# Autodesk Inventor assembly: LIDAR-Mapping-Assembly
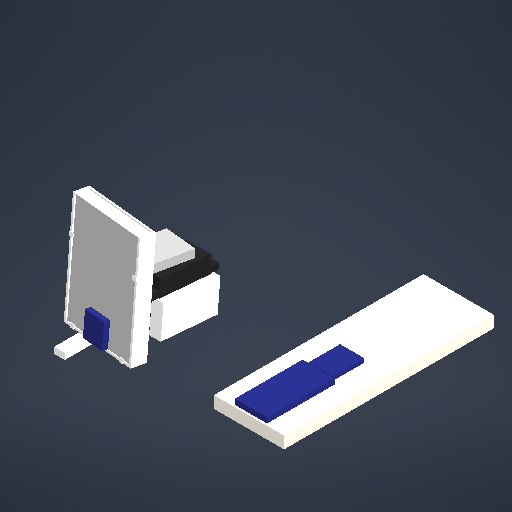
[picture p0: Inventor's stored thumbnail of the model, 512x512]
Saved by Autodesk Inventor 2025 (Build 290162000, 162)
## iProperties
Created: 2024-04-23
Part Number: LIDAR-Mapping-Assembly
Document SubType Name: Assembly
Designer: conno
Author: conno
## Documents named in this file (7)
- D:\OneDrive\Connor Sempf\Georgia Tech\Classes\Semester 6 - Spring 2024\ECE 4180 - Embedded Systems Design\Project\Project Files\3D Models\Assemblies\LIDAR-Mapper.iam
- D:\OneDrive\Connor Sempf\Georgia Tech\Classes\Semester 6 - Spring 2024\ECE 4180 - Embedded Systems Design\Project\Project Files\3D Models\Parts\Project Components\Servo.ipt
- D:\OneDrive\Connor Sempf\Georgia Tech\Classes\Semester 6 - Spring 2024\ECE 4180 - Embedded Systems Design\Project\Project Files\3D Models\Parts\3D Printed Parts\HorizontalRotationServoHolder.ipt
- D:\OneDrive\Connor Sempf\Georgia Tech\Classes\Semester 6 - Spring 2024\ECE 4180 - Embedded Systems Design\Project\Project Files\3D Models\Parts\3D Printed Parts\VerticalRotationServoHolder.ipt
- D:\OneDrive\Connor Sempf\Georgia Tech\Classes\Semester 6 - Spring 2024\ECE 4180 - Embedded Systems Design\Project\Project Files\3D Models\Parts\3D Printed Parts\BreadboardHousing.ipt
- D:\OneDrive\Connor Sempf\Georgia Tech\Classes\Semester 6 - Spring 2024\ECE 4180 - Embedded Systems Design\Project\Project Files\3D Models\Parts\Project Components\30RowBreadboard.ipt
- D:\OneDrive\Connor Sempf\Georgia Tech\Classes\Semester 6 - Spring 2024\ECE 4180 - Embedded Systems Design\Project\Project Files\3D Models\Parts\Project Components\63RowBreadboard.ipt
## Components (7 placed, 6 different names)
1. HorizontalRotationServoHolder-Left — Mate:5, Flush:6, Flush:7, Flush:18, Flush:19, Mate:16
2. VerticalRotationServoHolder:1 — Mate:6, Mate:7, Mate:8, Mate:9, Tangent:1, Tangent:2, Mate:13, Flush:10
3. Servo:2 — Mate:5, Flush:6, Flush:7, Mate:6, Tangent:1, Tangent:2
4. Servo:3 — Mate:7, Mate:8, Mate:9, Mate:12, Tangent:3, Tangent:4
5. BreadboardHousing:1 — Mate:12, Mate:13, Flush:10, Tangent:3, Tangent:4, Mate:14, Flush:17, Mate:15
6. 30RowBreadboard:1 — Mate:14, Flush:17, Mate:15
7. 63RowBreadboard:1 — Flush:18, Flush:19, Mate:16
## Relationships (20: Mate 10, Flush 6, Tangent 4)
- Mate:5: HorizontalRotationServoHolder-Left ↔ Servo:2
- Flush:6: HorizontalRotationServoHolder-Left ↔ Servo:2
- Flush:7: HorizontalRotationServoHolder-Left ↔ Servo:2
- Mate:6: VerticalRotationServoHolder:1 ↔ Servo:2
- Mate:7: VerticalRotationServoHolder:1 ↔ Servo:3
- Mate:8 (0.7937 mm): VerticalRotationServoHolder:1 ↔ Servo:3
- Mate:9 (0.7937 mm): VerticalRotationServoHolder:1 ↔ Servo:3
- Tangent:1: VerticalRotationServoHolder:1 ↔ Servo:2
- Tangent:2: VerticalRotationServoHolder:1 ↔ Servo:2
- Mate:12: Servo:3 ↔ BreadboardHousing:1
- Mate:13 (6.35 mm): VerticalRotationServoHolder:1 ↔ BreadboardHousing:1
- Flush:10: VerticalRotationServoHolder:1 ↔ BreadboardHousing:1
- Tangent:3 (19.05 mm): Servo:3 ↔ BreadboardHousing:1
- Tangent:4 (0.7937 mm): Servo:3 ↔ BreadboardHousing:1
- Mate:14: BreadboardHousing:1 ↔ 30RowBreadboard:1
- Flush:17: BreadboardHousing:1 ↔ 30RowBreadboard:1
- Mate:15: BreadboardHousing:1 ↔ 30RowBreadboard:1
- Flush:18: HorizontalRotationServoHolder-Left ↔ 63RowBreadboard:1
- Flush:19: HorizontalRotationServoHolder-Left ↔ 63RowBreadboard:1
- Mate:16 (76.2 mm): HorizontalRotationServoHolder-Left ↔ 63RowBreadboard:1
